# Autodesk Inventor assembly: Finger
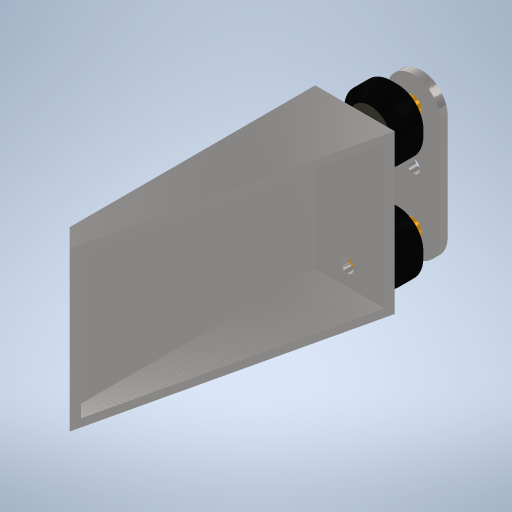
[picture p0: Inventor's stored thumbnail of the model, 512x512]
Saved by Autodesk Inventor 2024.2 (Build 282272000, 272)
## iProperties
Created: 2025-04-11
Part Number: Finger
Document SubType Name: Assembly
Designer: Admin
Author: Admin
## Documents named in this file (4)
- C:\Users\Admin\Documents\GitHub\GripperPropuesto\Assemblies\Finger.iam
- C:\Users\Admin\Documents\GitHub\GripperPropuesto\Assemblies\BearingWithInsert.iam
- C:\Users\Admin\Documents\GitHub\GripperPropuesto\AuxiliarPieces\FingerSupport\FingerSupport.ipt
- C:\Users\Admin\Documents\GitHub\GripperPropuesto\AuxiliarPieces\Claw\Claw.ipt
## Components (4 placed, 3 different names)
1. BearingWithInsert:1 [sub-assembly] — Mate:1, Mate:2, Mate:6
2. BearingWithInsert:2 [sub-assembly] — Mate:3, Mate:4, Mate:5, Mate:7
3. FingerSupport:1 — Mate:1, Mate:2, Mate:3, Mate:4
4. Claw:1 — Mate:5, Mate:6, Mate:7
## Relationships (7: Mate 7)
- Mate:1: BearingWithInsert:1 ↔ FingerSupport:1
- Mate:2: BearingWithInsert:1 ↔ FingerSupport:1
- Mate:3: BearingWithInsert:2 ↔ FingerSupport:1
- Mate:4: BearingWithInsert:2 ↔ FingerSupport:1
- Mate:5: BearingWithInsert:2 ↔ Claw:1
- Mate:6: BearingWithInsert:1 ↔ Claw:1
- Mate:7: BearingWithInsert:2 ↔ Claw:1
